# Autodesk Inventor assembly: BackUpperLink
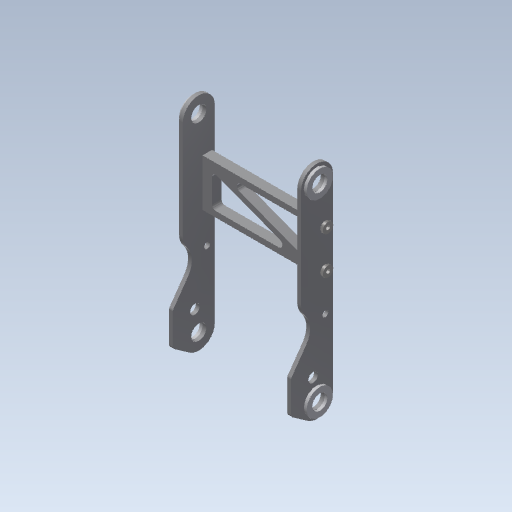
[picture p0: Inventor's stored thumbnail of the model, 512x512]
Saved by Autodesk Inventor 2020 (Build 240168000, 168)
## iProperties
Created: 2016-08-23
Part Number: BackUpperLink
Material: 一般
Document SubType Name: Assembly
Designer: hiro
Mass: 27.0677 g
Surface Area: 148.123 cm^2
Volume: 12.1706 cm^3
Density: 2.22402 g/cm^3
Author: hiro
## Documents named in this file (5)
- C:\Users\Masato\Desktop\OpenPlatform_ver3_0 - Ver4_1branch\LowerBody\Link\BackUpperLink.iam
- C:\Users\Masato\Desktop\OpenPlatform_ver3_0 - Ver4_1branch\LowerBody\Link\BackLink_diagonal.ipt
- C:\Users\Masato\Desktop\OpenPlatform_ver3_0 - Ver4_1branch\Ready_Made\Screw\M3-6.ipt
- C:\Users\Masato\Desktop\OpenPlatform_ver3_0 - Ver4_1branch\LowerBody\Link\BackLink_frame.ipt
- C:\Users\Masato\Desktop\OpenPlatform_ver3_0 - Ver4_1branch\Ready_Made\TT-0814-15.ipt
## Components (11 placed, 4 different names)
1. BackLink_diagonal:1 — 挿入:31, 挿入:32, 挿入:33, 挿入:34, フラッシュ:1, メイト:1
2. M3-6:1 — 挿入:38
3. M3-6:2 — 挿入:37
4. M3-6:3 — 挿入:41
5. M3-6:4 — 挿入:40
6. BackLink_frame:1 — 挿入:33, 挿入:34, 挿入:37, 挿入:38, 挿入:42, 挿入:45
7. BackLink_frame:2 — 挿入:31, 挿入:32, 挿入:40, 挿入:41, フラッシュ:2, 挿入:43, 挿入:44
8. TT-0814-15:1 — 挿入:42
9. TT-0814-15:2 — 挿入:43
10. TT-0814-15:3 — 挿入:44
11. TT-0814-15:4 — 挿入:45
## Relationships (15: Insert 12, Flush 2, Mate 1)
- 挿入:31 [Insert]: BackLink_diagonal:1 ↔ BackLink_frame:2
- 挿入:32 [Insert]: BackLink_diagonal:1 ↔ BackLink_frame:2
- 挿入:33 [Insert]: BackLink_diagonal:1 ↔ BackLink_frame:1
- 挿入:34 [Insert]: BackLink_diagonal:1 ↔ BackLink_frame:1
- 挿入:37 [Insert]: M3-6:2 ↔ BackLink_frame:1
- 挿入:38 [Insert]: M3-6:1 ↔ BackLink_frame:1
- 挿入:40 [Insert]: M3-6:4 ↔ BackLink_frame:2
- 挿入:41 [Insert]: M3-6:3 ↔ BackLink_frame:2
- フラッシュ:1 [Flush]: BackLink_diagonal:1
- メイト:1 [Mate]: BackLink_diagonal:1
- フラッシュ:2 [Flush]: BackLink_frame:2
- 挿入:42 [Insert]: BackLink_frame:1 ↔ TT-0814-15:1
- 挿入:43 [Insert]: BackLink_frame:2 ↔ TT-0814-15:2
- 挿入:44 [Insert]: BackLink_frame:2 ↔ TT-0814-15:3
- 挿入:45 [Insert]: BackLink_frame:1 ↔ TT-0814-15:4
